# Autodesk Inventor assembly: sensorcasing
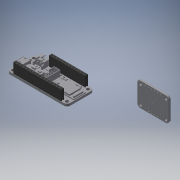
[picture p0: Inventor's stored thumbnail of the model, 180x180]
Saved by Autodesk Inventor 2017 (Build 210142000, 142)
## iProperties
Part Number: sensorcasing
Material: Generisch
Document SubType Name: Assembly
Designer: Enno
Author: Enno
## Documents named in this file (5)
- C:\Users\Enno\Desktop\IMU_Motion_Classification\Adafruit_Feather\CAD\sensorcasing.iam
- C:\Users\Enno\Desktop\IMU_Motion_Classification\Adafruit_Feather\CAD\adafruit-bno055-1.snapshot.9\Adafruit BNO055\Adafruit_BNO055_AP203.ipt
- C:\Users\Enno\Desktop\IMU_Motion_Classification\Adafruit_Feather\CAD\adafruit-4062-nrf52830-feather-1.snapshot.2\4062-nRF52830-Feather.ipt
- C:\Users\Enno\Desktop\IMU_Motion_Classification\Adafruit_Feather\CAD\stiftleiste_male-1.snapshot.20\Weib\Gerade\BuchsenLeiste16.iam
- C:\Users\Enno\Desktop\IMU_Motion_Classification\Adafruit_Feather\CAD\stiftleiste_male-1.snapshot.20\Weib\Gerade\BuchsenLeiste12.iam
## Components (4 placed, 4 different names)
1. Adafruit_BNO055_AP203:1
2. 4062-nRF52830-Feather:1 — Passend:1, Passend:2, Passend:3, Passend:4, Passend:5, Passend:6
3. BuchsenLeiste16:1 [sub-assembly] — Passend:1, Passend:2, Passend:3
4. BuchsenLeiste12:1 [sub-assembly] — Passend:4, Passend:5, Passend:6
## Relationships (6: Mate 6)
- Passend:1 [Mate]: 4062-nRF52830-Feather:1 ↔ BuchsenLeiste16:1
- Passend:2 [Mate]: 4062-nRF52830-Feather:1 ↔ BuchsenLeiste16:1
- Passend:3 [Mate]: 4062-nRF52830-Feather:1 ↔ BuchsenLeiste16:1
- Passend:4 [Mate]: 4062-nRF52830-Feather:1 ↔ BuchsenLeiste12:1
- Passend:5 [Mate]: 4062-nRF52830-Feather:1 ↔ BuchsenLeiste12:1
- Passend:6 [Mate]: 4062-nRF52830-Feather:1 ↔ BuchsenLeiste12:1
